# Autodesk Inventor assembly: 3136 1133 80
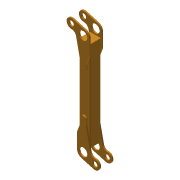
[picture p0: Inventor's stored thumbnail of the model, 180x180]
Saved by Autodesk Inventor 2022 Beta2 (Build 260130000, 130) ContinuousBuild 0
## iProperties
Shininess: 64.0
Length Units: 11269
Angle Units: 11279
Time Units: 11290
Mass Units: 11283
Length Display Precision: 3
Angle Display Precision: 2
Compacted: True
Created: 2003-04-13
Part Number: 3136 1133 80
Document SubType Name: Assembly
Designer: Uffe Bak
Density: 0.0
Volumn: 0.0
Area: 0.0
PropertySet Name: Model Information
Control State: 0
Master: False
Checked Out: False
Author: Uffe Bak
## Documents named in this file (4)
- C:\Autodesk Inventor 2021 Intro Practice Files\BOM\3136 1133 80.iam
- C:\Autodesk Inventor 2021 Intro Practice Files\BOM\3136 1094 43.ipt
- C:\Autodesk Inventor 2021 Intro Practice Files\BOM\3136 1133 81.ipt
- C:\Autodesk Inventor 2021 Intro Practice Files\BOM\3136 1094 58.ipt
## Components (7 placed, 3 different names)
1. 3136 1094 43:1 — Flush:1, Mate:1, Mate:2, Mate:3, Mate:5, Mate:6, Mate:7, Angle:1, Mate:8, Mate:10, Mate:11, Mate:12, Mate:13, Flush:4, Mate:14
2. 3136 1133 81:1 — Flush:1, Mate:1, Mate:2, Mate:4, Flush:2
3. 3136 1133 81:2 — Mate:3, Mate:4, Flush:2
4. 3136 1133 81:3 — Mate:5, Mate:6, Mate:7, Angle:1, Mate:9, Flush:3
5. 3136 1133 81:4 — Mate:8, Mate:9, Flush:3
6. 3136 1094 58:1 — Mate:10, Mate:11, Mate:12
7. 3136 1094 58:2 — Mate:13, Flush:4, Mate:14
## Relationships (19: Mate 14, Flush 4, Angle 1)
- Flush:1: 3136 1094 43:1 ↔ 3136 1133 81:1
- Mate:1: 3136 1094 43:1 ↔ 3136 1133 81:1
- Mate:2 (40 mm): 3136 1094 43:1 ↔ 3136 1133 81:1
- Mate:3: 3136 1094 43:1 ↔ 3136 1133 81:2
- Mate:4: 3136 1133 81:1 ↔ 3136 1133 81:2
- Flush:2: 3136 1133 81:1 ↔ 3136 1133 81:2
- Mate:5: 3136 1094 43:1 ↔ 3136 1133 81:3
- Mate:6 (40 mm): 3136 1094 43:1 ↔ 3136 1133 81:3
- Mate:7: 3136 1094 43:1 ↔ 3136 1133 81:3
- Angle:1 (0 deg): 3136 1094 43:1 ↔ 3136 1133 81:3
- Mate:8: 3136 1094 43:1 ↔ 3136 1133 81:4
- Mate:9: 3136 1133 81:3 ↔ 3136 1133 81:4
- Flush:3: 3136 1133 81:3 ↔ 3136 1133 81:4
- Mate:10: 3136 1094 43:1 ↔ 3136 1094 58:1
- Mate:11: 3136 1094 43:1 ↔ 3136 1094 58:1
- Mate:12: 3136 1094 43:1 ↔ 3136 1094 58:1
- Mate:13: 3136 1094 43:1 ↔ 3136 1094 58:2
- Flush:4: 3136 1094 43:1 ↔ 3136 1094 58:2
- Mate:14: 3136 1094 43:1 ↔ 3136 1094 58:2
